# Autodesk Inventor assembly: Assembly_cube_StormChip_v4
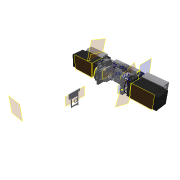
[picture p0: Inventor's stored thumbnail of the model, 180x180]
Saved by Autodesk Inventor 2019 (Build 230136000, 136)
## iProperties
Created: 2018-06-27
Part Number: Assembly_cube_StormChip_v4
Material: Generisch
Document SubType Name: Assembly
Designer: diederichbenedict
Author: diederichbenedict
## Documents named in this file (17)
- C:\Users\diederichbenedict\Dropbox\Dokumente\Promotion\PROJECTS\STORMoChip\INVENTOR\Workspaces\Arbeitsbereich\10_Cube_Base\Assembly_cube_StormChip_v4.iam
- C:\Users\diederichbenedict\Dropbox\Dokumente\Promotion\PROJECTS\STORMoChip\INVENTOR\Workspaces\Arbeitsbereich\10_Cube_Base\10_Cube_3x_v0.ipt
- C:\Users\diederichbenedict\Dropbox\Dokumente\Promotion\PROJECTS\STORMoChip\INVENTOR\Workspaces\Arbeitsbereich\10_Cube_Base\10_Lid_el_3x_v0.ipt
- C:\Users\diederichbenedict\Dropbox\Dokumente\Promotion\PROJECTS\STORMoChip\INVENTOR\Workspaces\Arbeitsbereich\10_Cube_Base\LASER_640nm.ipt
- C:\Users\diederichbenedict\Dropbox\Dokumente\Promotion\PROJECTS\STORMoChip\INVENTOR\Workspaces\Arbeitsbereich\10_Cube_Base\40_XYZ_Adapter_Flattener.ipt
- C:\Users\diederichbenedict\Dropbox\Dokumente\Promotion\PROJECTS\STORMoChip\INVENTOR\Workspaces\Arbeitsbereich\10_Cube_Base\00_dSTORM_Chip.ipt
- C:\Users\diederichbenedict\Dropbox\Dokumente\Promotion\PROJECTS\STORMoChip\INVENTOR\Workspaces\Arbeitsbereich\10_Cube_Base\Raman2Go_ProbenhalterXY-Verstellung_mit_Adapterplatten.iam
- C:\Users\diederichbenedict\Dropbox\Dokumente\Promotion\PROJECTS\STORMoChip\INVENTOR\Workspaces\Arbeitsbereich\10_Cube_Base\20_Base_STORMchip_doublesided_railsystem.ipt
- C:\Users\diederichbenedict\Dropbox\Dokumente\Promotion\PROJECTS\STORMoChip\INVENTOR\Workspaces\Arbeitsbereich\10_Cube_Base\CP02_M-Step.ipt
- C:\Users\diederichbenedict\Dropbox\Dokumente\Promotion\PROJECTS\STORMoChip\INVENTOR\Workspaces\Arbeitsbereich\10_Cube_Base\00_160mm_Rod_Thorlabs.ipt
- C:\Users\diederichbenedict\Dropbox\Dokumente\Promotion\PROJECTS\STORMoChip\INVENTOR\Workspaces\Arbeitsbereich\10_Cube_Base\20_Adapter_Laser_Thorlabs.ipt
- C:\Users\diederichbenedict\Dropbox\Dokumente\Promotion\PROJECTS\STORMoChip\INVENTOR\Workspaces\Arbeitsbereich\10_Cube_Base\00_40mm_Rod_Thorlabs.ipt
- C:\Users\diederichbenedict\Dropbox\Dokumente\Promotion\PROJECTS\STORMoChip\INVENTOR\Workspaces\Arbeitsbereich\10_Cube_Base\Assembly_Lens_XY_Translator.iam
- C:\Users\diederichbenedict\Dropbox\Dokumente\Promotion\PROJECTS\STORMoChip\INVENTOR\Workspaces\Arbeitsbereich\10_Cube_Base\Assembly_Lens_Thorlabs_Mount_KES400_Bluraylasermount.iam
- C:\Users\diederichbenedict\Dropbox\Dokumente\Promotion\PROJECTS\STORMoChip\INVENTOR\Workspaces\Arbeitsbereich\20_Base_STORMchip_doublesided_railsystem_Laser.ipt
- C:\Users\diederichbenedict\Dropbox\Dokumente\Promotion\PROJECTS\STORMoChip\INVENTOR\Workspaces\Arbeitsbereich\10_Cube_Base\00_KES400_Bluray_Lens.ipt
- C:\Users\diederichbenedict\Dropbox\Dokumente\Promotion\PROJECTS\STORMoChip\INVENTOR\Workspaces\Arbeitsbereich\00_Laser_coupling.ipt
## Components (21 placed, 16 different names)
1. 10_Cube_3x_v0:1 — Einfügen:1, Einfügen:2, Passend:1, Winkel:2, Winkel:3
2. 10_Lid_el_3x_v0:1 — Einfügen:1, Einfügen:2
3. 40_XYZ_Adapter_Flattener:1
4. 00_dSTORM_Chip:1 — Passend:1, Winkel:3
5. 00_dSTORM_Chip:2 — Winkel:2, Mate:20
6. 20_Base_STORMchip_doublesided_railsystem:1 — Angle:10, Mate:14, Mate:15, Mate:16, Angle:11, Angle:13, Flush:9, Flush:10
7. CP02_M-Step:1 — Angle:13, Flush:9, Flush:10, Mate:18, Mate:19, Mate:25, Mate:26
8. Raman2Go_ProbenhalterXY-Verstellung_mit_Adapterplatten:2 [sub-assembly] — Angle:10, Mate:14, Mate:15, Mate:20
9. LASER_640nm:3 — Mate:16, Angle:11, Flush:12, Flush:13, Flush:14, Flush:15, Mate:34
10. 00_160mm_Rod_Thorlabs:1 — Mate:18, Mate:24, Mate:31
11. 00_160mm_Rod_Thorlabs:2 — Mate:19, Mate:23, Mate:32
12. 20_Adapter_Laser_Thorlabs:1 — Flush:12
13. 00_40mm_Rod_Thorlabs:1 — Mate:25, Insert:4
14. 00_40mm_Rod_Thorlabs:2 — Mate:26, Insert:3
15. Assembly_Lens_XY_Translator:1 [sub-assembly] — Mate:23, Mate:24, Mate:36, Angle:15
16. Assembly_Lens_Thorlabs_Mount_KES400_Bluraylasermount:1 [sub-assembly] — Insert:3, Insert:4, Flush:17, Flush:18
17. 20_Base_STORMchip_doublesided_railsystem_Laser:1 — Flush:13, Flush:14, Flush:15
18. 20_Base_STORMchip_doublesided_railsystem_Laser:2 — Mate:31, Mate:32, Mate:33, Flush:16
19. LASER_640nm:4 — Mate:33, Flush:16, Mate:34, Mate:37
20. 00_KES400_Bluray_Lens:1 — Mate:36, Mate:37, Angle:15
21. 00_Laser_coupling:1 — Flush:17, Flush:18
## Relationships (39: Mate 19, Flush 9, Angle 7, Insert 4)
- Einfügen:1 [Insert]: 10_Cube_3x_v0:1 ↔ 10_Lid_el_3x_v0:1
- Einfügen:2 [Insert]: 10_Cube_3x_v0:1 ↔ 10_Lid_el_3x_v0:1
- Passend:1 [Mate]: 10_Cube_3x_v0:1 ↔ 00_dSTORM_Chip:1
- Winkel:2 [Angle] (0 deg): 10_Cube_3x_v0:1 ↔ 00_dSTORM_Chip:2
- Winkel:3 [Angle] (0 deg): 10_Cube_3x_v0:1 ↔ 00_dSTORM_Chip:1
- Angle:10 (180 deg): 20_Base_STORMchip_doublesided_railsystem:1 ↔ Raman2Go_ProbenhalterXY-Verstellung_mit_Adapterplatten:2
- Mate:14: 20_Base_STORMchip_doublesided_railsystem:1 ↔ Raman2Go_ProbenhalterXY-Verstellung_mit_Adapterplatten:2
- Mate:15: 20_Base_STORMchip_doublesided_railsystem:1 ↔ Raman2Go_ProbenhalterXY-Verstellung_mit_Adapterplatten:2
- Mate:16: 20_Base_STORMchip_doublesided_railsystem:1 ↔ LASER_640nm:3
- Angle:11 (0 deg): 20_Base_STORMchip_doublesided_railsystem:1 ↔ LASER_640nm:3
- Angle:13 (0 deg): 20_Base_STORMchip_doublesided_railsystem:1 ↔ CP02_M-Step:1
- Flush:9 (-0.32 mm): 20_Base_STORMchip_doublesided_railsystem:1 ↔ CP02_M-Step:1
- Flush:10 (1 mm): 20_Base_STORMchip_doublesided_railsystem:1 ↔ CP02_M-Step:1
- Mate:18: CP02_M-Step:1 ↔ 00_160mm_Rod_Thorlabs:1
- Mate:19: CP02_M-Step:1 ↔ 00_160mm_Rod_Thorlabs:2
- Flush:12: LASER_640nm:3 ↔ 20_Adapter_Laser_Thorlabs:1
- Mate:20: 00_dSTORM_Chip:2 ↔ Raman2Go_ProbenhalterXY-Verstellung_mit_Adapterplatten:2
- Mate:23: 00_160mm_Rod_Thorlabs:2 ↔ Assembly_Lens_XY_Translator:1
- Mate:24: 00_160mm_Rod_Thorlabs:1 ↔ Assembly_Lens_XY_Translator:1
- Mate:25: CP02_M-Step:1 ↔ 00_40mm_Rod_Thorlabs:1
- Mate:26: CP02_M-Step:1 ↔ 00_40mm_Rod_Thorlabs:2
- Insert:3: 00_40mm_Rod_Thorlabs:2 ↔ Assembly_Lens_Thorlabs_Mount_KES400_Bluraylasermount:1
- Insert:4: 00_40mm_Rod_Thorlabs:1 ↔ Assembly_Lens_Thorlabs_Mount_KES400_Bluraylasermount:1
- [Mate]: LASER_640nm:3 ↔ Assembly_Lens_Thorlabs_Mount_KES400_Bluraylasermount:1
- [Angle] (0 deg): LASER_640nm:3 ↔ Assembly_Lens_Thorlabs_Mount_KES400_Bluraylasermount:1
- Flush:13: LASER_640nm:3 ↔ 20_Base_STORMchip_doublesided_railsystem_Laser:1
- Flush:14: LASER_640nm:3 ↔ 20_Base_STORMchip_doublesided_railsystem_Laser:1
- Flush:15: LASER_640nm:3 ↔ 20_Base_STORMchip_doublesided_railsystem_Laser:1
- Mate:31: 00_160mm_Rod_Thorlabs:1 ↔ 20_Base_STORMchip_doublesided_railsystem_Laser:2
- Mate:32: 00_160mm_Rod_Thorlabs:2 ↔ 20_Base_STORMchip_doublesided_railsystem_Laser:2
- Mate:33: 20_Base_STORMchip_doublesided_railsystem_Laser:2 ↔ LASER_640nm:4
- Flush:16: 20_Base_STORMchip_doublesided_railsystem_Laser:2 ↔ LASER_640nm:4
- Mate:34: LASER_640nm:3 ↔ LASER_640nm:4
- [Mate]: Assembly_Lens_XY_Translator:1 ↔ LASER_640nm:4
- Mate:36: Assembly_Lens_XY_Translator:1 ↔ 00_KES400_Bluray_Lens:1
- Mate:37: LASER_640nm:4 ↔ 00_KES400_Bluray_Lens:1
- Angle:15 (180 deg): Assembly_Lens_XY_Translator:1 ↔ 00_KES400_Bluray_Lens:1
- Flush:17: Assembly_Lens_Thorlabs_Mount_KES400_Bluraylasermount:1 ↔ 00_Laser_coupling:1
- Flush:18 (4 mm): Assembly_Lens_Thorlabs_Mount_KES400_Bluraylasermount:1 ↔ 00_Laser_coupling:1
